# Autodesk Inventor assembly: A_Aft
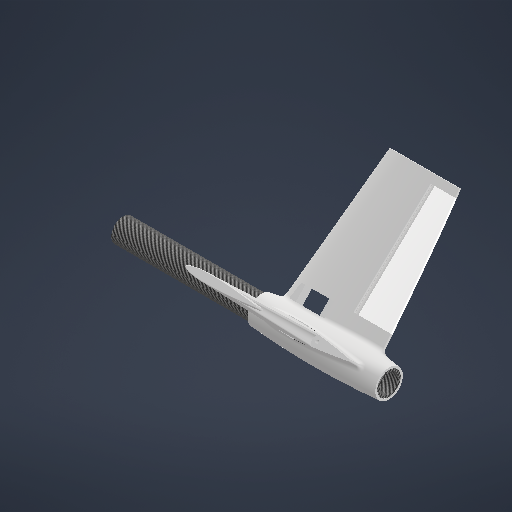
[picture p0: Inventor's stored thumbnail of the model, 512x512]
Saved by Autodesk Inventor 2026 (Build 300175000, 175)
## iProperties
Created: 2025-09-10
Part Number: A_Aft
Document SubType Name: Assembly
Designer: FAL
Author: FAL
## Documents named in this file (4)
- C:\Users\FAL\Projekte\Git\AIRBERT\CAD\Aft\A_Aft.iam
- C:\Users\FAL\Projekte\Git\AIRBERT\CAD\Aft\P_aft_V.ipt
- C:\Users\FAL\Projekte\Git\AIRBERT\CAD\Aft\P_aft_V_rudder.ipt
- C:\Users\FAL\Projekte\Git\AIRBERT\CAD\Aft\P_Carbon_Pipe_Back.ipt
## Components (3 placed, 3 different names)
1. P_aft_V:1 — Fluchtend:1, Fluchtend:2, Fluchtend:3, Fluchtend:10
2. P_aft_V_rudder:1 — Fluchtend:4, Fluchtend:5, Fluchtend:6
3. P_Carbon_Pipe_Back:1 — Fluchtend:8, Fluchtend:9, Fluchtend:10
## Relationships (9: Flush 9)
- Fluchtend:1 [Flush]: P_aft_V:1
- Fluchtend:2 [Flush]: P_aft_V:1
- Fluchtend:3 [Flush]: P_aft_V:1
- Fluchtend:4 [Flush]: P_aft_V_rudder:1
- Fluchtend:5 [Flush]: P_aft_V_rudder:1
- Fluchtend:6 [Flush]: P_aft_V_rudder:1
- Fluchtend:8 [Flush]: P_Carbon_Pipe_Back:1
- Fluchtend:9 [Flush]: P_Carbon_Pipe_Back:1
- Fluchtend:10 [Flush]: P_aft_V:1 ↔ P_Carbon_Pipe_Back:1
